# Autodesk Inventor assembly: Bumper Assembly1 (24x28 robot)
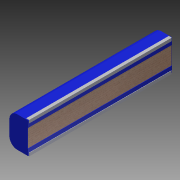
[picture p0: Inventor's stored thumbnail of the model, 180x180]
Saved by Autodesk Inventor 2013 (Build 170138000, 138)
## iProperties
Created: 2013-01-06
Part Number: Bumper Assembly1 (24x28 robot)
Document SubType Name: Assembly
Designer: Moses
Mass: 1437.55 g
Surface Area: 12857.4 cm^2
Volume: 6466.78 cm^3
Density: 0.222298 g/cm^3
Author: Moses
## Documents named in this file (5)
- C:\Users\Moses\Documents\GitHub\frc2013CAD\Robot Chassis and Drivetrain\Chassis\Bumpers\Bumper Assembly1 (24x28 robot).iam
- C:\Users\Moses\Documents\GitHub\frc2013CAD\Robot Chassis and Drivetrain\Chassis\Bumpers\Bumper Wood Backing Part1 (24x28 robot).ipt
- C:\Users\Moses\Documents\GitHub\frc2013CAD\Robot Chassis and Drivetrain\Chassis\Bumpers\Bumper Cover Part1 (24x28 robot).ipt
- C:\Users\Moses\Documents\GitHub\frc2013CAD\Robot Chassis and Drivetrain\Chassis\Bumpers\Bumper Metal Edge Part1 (24x28 robot).ipt
- C:\Users\Moses\Documents\GitHub\frc2013CAD\Robot Chassis and Drivetrain\Chassis\Bumpers\Pool Noodle Part1 (24x28 robot).ipt
## Components (6 placed, 4 different names)
1. Bumper Wood Backing Part1 (24x28 robot):1 — Tangent:1, Tangent:2, Flush:2, Flush:3, Tangent:4, Mate:2
2. Pool Noodle Part1 (24x28 robot):1 — Tangent:1, Tangent:3, Flush:1
3. Pool Noodle Part1 (24x28 robot):2 — Tangent:2, Tangent:3, Flush:1, Flush:2, Tangent:4, Mate:1, Tangent:5
4. Bumper Cover Part1 (24x28 robot):1 — Flush:3, Mate:1, Mate:2, Tangent:5, Mate:3, Mate:4, Mate:5, Mate:6, Flush:5
5. Bumper Metal Edge Part1 (24x28 robot):1 — Mate:5, Mate:6, Flush:4, Flush:5
6. Bumper Metal Edge Part1 (24x28 robot):2 — Mate:3, Mate:4, Flush:4
## Relationships (16: Mate 6, Tangent 5, Flush 5)
- Tangent:1: Bumper Wood Backing Part1 (24x28 robot):1 ↔ Pool Noodle Part1 (24x28 robot):1
- Tangent:2: Bumper Wood Backing Part1 (24x28 robot):1 ↔ Pool Noodle Part1 (24x28 robot):2
- Tangent:3: Pool Noodle Part1 (24x28 robot):1 ↔ Pool Noodle Part1 (24x28 robot):2
- Flush:1: Pool Noodle Part1 (24x28 robot):1 ↔ Pool Noodle Part1 (24x28 robot):2
- Flush:2: Bumper Wood Backing Part1 (24x28 robot):1 ↔ Pool Noodle Part1 (24x28 robot):2
- Flush:3: Bumper Wood Backing Part1 (24x28 robot):1 ↔ Bumper Cover Part1 (24x28 robot):1
- Tangent:4: Bumper Wood Backing Part1 (24x28 robot):1 ↔ Pool Noodle Part1 (24x28 robot):2
- Mate:1: Pool Noodle Part1 (24x28 robot):2 ↔ Bumper Cover Part1 (24x28 robot):1
- Mate:2: Bumper Wood Backing Part1 (24x28 robot):1 ↔ Bumper Cover Part1 (24x28 robot):1
- Tangent:5: Pool Noodle Part1 (24x28 robot):2 ↔ Bumper Cover Part1 (24x28 robot):1
- Mate:3: Bumper Cover Part1 (24x28 robot):1 ↔ Bumper Metal Edge Part1 (24x28 robot):2
- Mate:4: Bumper Cover Part1 (24x28 robot):1 ↔ Bumper Metal Edge Part1 (24x28 robot):2
- Mate:5: Bumper Cover Part1 (24x28 robot):1 ↔ Bumper Metal Edge Part1 (24x28 robot):1
- Mate:6: Bumper Cover Part1 (24x28 robot):1 ↔ Bumper Metal Edge Part1 (24x28 robot):1
- Flush:4: Bumper Metal Edge Part1 (24x28 robot):1 ↔ Bumper Metal Edge Part1 (24x28 robot):2
- Flush:5 (3.175 mm): Bumper Cover Part1 (24x28 robot):1 ↔ Bumper Metal Edge Part1 (24x28 robot):1
